# Autodesk Inventor assembly: Holder
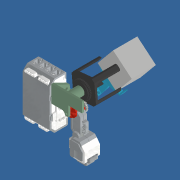
[picture p0: Inventor's stored thumbnail of the model, 180x180]
Saved by Autodesk Inventor 2020 (Build 240168000, 168)
## iProperties
Created: 2019-12-14
Part Number: Holder
Document SubType Name: Assembly
Designer: Jack
Author: Jack
## Documents named in this file (8)
- D:\Code\Python\EV3_Cuber\3D Model\Holder.iam
- D:\Code\Python\EV3_Cuber\3D Model\HolderGear.ipt
- D:\Code\Python\EV3_Cuber\3D Model\HolderShaft.ipt
- D:\Code\Python\EV3_Cuber\3D Model\Cube.ipt
- D:\Code\Python\EV3_Cuber\3D Model\Hand.ipt
- D:\Code\Python\EV3_Cuber\3D Model\MotorL.ipt
- D:\Code\Python\EV3_Cuber\3D Model\Brick.ipt
- D:\Code\Python\EV3_Cuber\3D Model\Gear 24.ipt
## Components (7 placed, 7 different names)
1. HolderShaft:1 — Mate:8, Mate:9, Mate:10, Angle:4, Rotational:3
2. HolderGear:1 — Angle:1, Angle:2, Mate:5, Mate:7, Flush:1, Rotational:3
3. Cube:1 — Angle:1, Angle:2, Mate:5, Mate:7, Angle:3, Mate:11, Mate:12
4. Hand:1 — Angle:3, Mate:11, Mate:12
5. MotorL:1 — Rotational:2, Mate:10, Angle:4
6. Brick:1 — Mate:8, Mate:9
7. Gear 24:1 — Rotational:2, Flush:1
## Relationships (14: Mate 7, Angle 4, RevoluteJoint 2, Flush 1)
- Angle:1 (0 deg): HolderGear:1 ↔ Cube:1
- Angle:2 (0 deg): HolderGear:1 ↔ Cube:1
- Mate:5 (0.5 mm): HolderGear:1 ↔ Cube:1
- Mate:7 (0.5 mm): HolderGear:1 ↔ Cube:1
- Mate:8: HolderShaft:1 ↔ Brick:1
- Mate:9: HolderShaft:1 ↔ Brick:1
- Rotational:2 [RevoluteJoint]: MotorL:1 ↔ Gear 24:1
- Flush:1: HolderGear:1 ↔ Gear 24:1
- Mate:10: HolderShaft:1 ↔ MotorL:1
- Angle:3 (0 deg): Cube:1 ↔ Hand:1
- Mate:11 (0.5 mm): Cube:1 ↔ Hand:1
- Mate:12 (-14.5 mm): Cube:1 ↔ Hand:1
- Angle:4 (0 deg): HolderShaft:1 ↔ MotorL:1
- Rotational:3 [RevoluteJoint]: HolderShaft:1 ↔ HolderGear:1
